# Autodesk Inventor assembly: V Wheel - Eccentric Spacer - Bolt v2
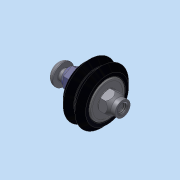
[picture p0: Inventor's stored thumbnail of the model, 180x180]
Saved by Autodesk Inventor 2013 (Build 170138000, 138)
## iProperties
Created: 2013-06-21
Part Number: V Wheel - Eccentric Spacer - Bolt v2
Document SubType Name: Assembly
Designer: Jon Hollander
Author: Jon Hollander
## Documents named in this file (5)
- D:\Dropbox\Research\CAD Library\v-slot\Part Assemblies v2\V Wheel - Eccentric Spacer - Bolt\V Wheel - Eccentric Spacer - Bolt v2.iam
- D:\Dropbox\Research\CAD Library\v-slot\V Wheel and Bearings.iam
- C:\Users\Work\Documents\Inventor\Content Center Files\R2013\en-US\ANSI B18.16.3M(2)\ANSI B18.16.3M - Property Class 5 and 10 - Metric M5 x 0.8 Top Insert Type.ipt
- C:\Users\Work\Documents\Inventor\Content Center Files\R2013\en-US\ANSI B18.3.4M(1)\ANSI B18.3.4M - M5 x 0.8 x 25(2).ipt
- C:\Users\Work\Documents\Inventor\Content Center Files\R2013\en-US\Eccentric M5 Spacer\Eccentric M5 Spacer.ipt
## Components (4 placed, 4 different names)
1. Broached Hexagon Socket Button Head Cap Screw - Metric M5 x 0.8 x 25:1 — Mate:13, Mate:16
2. Eccentric M5 Spacer Eccentric M5 Spacer:1
3. V Wheel and Bearings:1 [sub-assembly] — Mate:16, Mate:17
4. Prevailing Torque Type Hex Nut - Steel Metric Property Class 5 and 10 - Metric M5 x 0.8 Top Insert Type:1 — Mate:13, Mate:17
## Relationships (6: Mate 6)
- [Mate]: Broached Hexagon Socket Button Head Cap Screw - Metric M5 x 0.8 x 25:1 ↔ Eccentric M5 Spacer Eccentric M5 Spacer:1
- Mate:13: Broached Hexagon Socket Button Head Cap Screw - Metric M5 x 0.8 x 25:1 ↔ Prevailing Torque Type Hex Nut - Steel Metric Property Class 5 and 10 - Metric M5 x 0.8 Top Insert Type:1
- [Mate] (3 mm): Broached Hexagon Socket Button Head Cap Screw - Metric M5 x 0.8 x 25:1 ↔ Eccentric M5 Spacer Eccentric M5 Spacer:1
- Mate:16: Broached Hexagon Socket Button Head Cap Screw - Metric M5 x 0.8 x 25:1 ↔ V Wheel and Bearings:1
- Mate:17: V Wheel and Bearings:1 ↔ Prevailing Torque Type Hex Nut - Steel Metric Property Class 5 and 10 - Metric M5 x 0.8 Top Insert Type:1
- [Mate]: Eccentric M5 Spacer Eccentric M5 Spacer:1 ↔ V Wheel and Bearings:1
